# Autodesk Inventor assembly: solenoid_swivel_brkt_plus
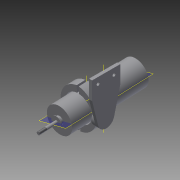
[picture p0: Inventor's stored thumbnail of the model, 180x180]
Saved by Autodesk Inventor 2015 (Build 190159000, 159)
## iProperties
Created: 2015-09-23
Part Number: solenoid_swivel_brkt_plus
Description: insert description/title
Document SubType Name: Assembly
Designer: francis
Author: francis
Part Category: insert part category and press enter to fill value
## Documents named in this file (3)
- C:\Users\francis\Documents\GitHub\CAD\solenoid_swivel_brkt_plus.iam
- C:\Users\francis\Documents\GitHub\CAD\swivel_brkt.iam
- C:\Users\francis\Documents\GitHub\CAD\solenoid assy.iam
## Components (2 placed, 2 different names)
1. swivel_brkt:1 [sub-assembly] — Cylindrical:1
2. solenoid assy:1 [sub-assembly] — Cylindrical:1
## Relationships (1: CylindricalJoint 1)
- Cylindrical:1: swivel_brkt:1 ↔ solenoid assy:1
